# Autodesk Inventor assembly: Assembly_Cube_Flashlight_v3
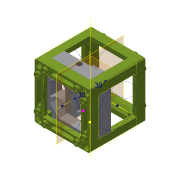
[picture p0: Inventor's stored thumbnail of the model, 180x180]
Saved by Autodesk Inventor 2019.4 (Build 234330000, 330)
## iProperties
Created: 2020-12-04
Part Number: Assembly_Cube_Flashlight_v3
Document SubType Name: Assembly
Designer: UC2
Author: UC2
## Documents named in this file (4)
- C:\Users\diederichbenedict\Dropbox\Dokumente\Promotion\PROJECTS\UC2\02_CAD\INVENTOR\uc2_v3\Assembly_Cube_Flexuremanipulator_zonly_v3.iam
- C:\Users\diederichbenedict\Dropbox\Dokumente\Promotion\PROJECTS\UC2\02_CAD\INVENTOR\uc2_v3\Assembly_Cube_empty_IM_v3.iam
- C:\Users\diederichbenedict\Dropbox\Dokumente\Promotion\PROJECTS\UC2\02_CAD\INVENTOR\uc2_v3\20_Cube_Inser_Flexuremanipulator_zonly_v3.ipt
- C:\Users\diederichbenedict\Downloads\00_mk8_nozzle_0.4STEP.ipt
## Components (3 placed, 3 different names)
1. Assembly_Cube_empty_IM_v3:1 [sub-assembly] — Mate:1, Flush:1, Flush:2
2. 20_Cube_Inser_Flexuremanipulator_zonly_v3:1 — Mate:1, Flush:1, Flush:2
3. 00_mk8_nozzle_0.4STEP:1
## Relationships (4: Flush 2, Mate 1, Insert 1)
- Mate:1: Assembly_Cube_empty_IM_v3:1 ↔ 20_Cube_Inser_Flexuremanipulator_zonly_v3:1
- Flush:1 (-0.05 mm): Assembly_Cube_empty_IM_v3:1 ↔ 20_Cube_Inser_Flexuremanipulator_zonly_v3:1
- Flush:2 (0.025 mm): Assembly_Cube_empty_IM_v3:1 ↔ 20_Cube_Inser_Flexuremanipulator_zonly_v3:1
- [Insert]: 20_Cube_Inser_Flexuremanipulator_zonly_v3:1 ↔ 00_mk8_nozzle_0.4STEP:1
